# Autodesk Inventor assembly: Frame_Gantry_Carrier_Reverse
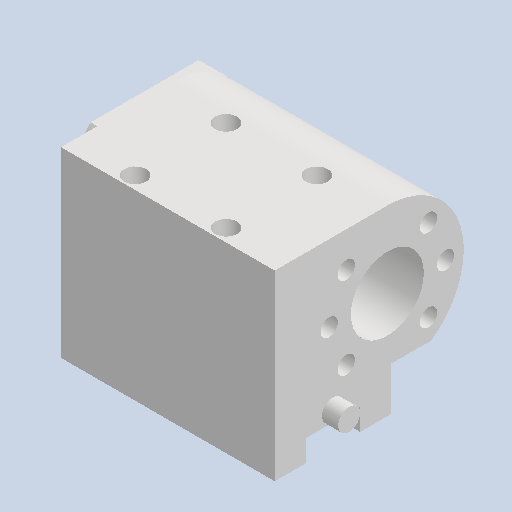
[picture p0: Inventor's stored thumbnail of the model, 512x512]
Saved by Autodesk Inventor 2023 (Build 270158000, 158)
## iProperties
Created: 2022-04-30
Part Number: Frame_Gantry_Carrier_Reverse
Document SubType Name: Assembly
Designer: plebbb
Author: plebbb
## Documents named in this file (4)
- D:\Users\plebbb\Desktop\CNC_Project\Frame_Gantry_Carrier_Reverse.iam
- D:\Users\plebbb\Desktop\CNC_Project\MGN15H-Carrier.ipt
- D:\Users\plebbb\Desktop\CNC_Project\SFU1204-Housing.ipt
- D:\Users\plebbb\Desktop\CNC_Project\X_Axis_Connector.ipt
## Components (3 placed, 3 different names)
1. MGN15H-Carrier:1
2. SFU1204-Housing:1
3. X_Axis_Connector:1
## Relationships (5: Mate 4, Angle 1)
- [Angle] (0 deg): MGN15H-Carrier:1 ↔ SFU1204-Housing:1
- [Mate]: MGN15H-Carrier:1 ↔ SFU1204-Housing:1
- [Mate]: MGN15H-Carrier:1 ↔ X_Axis_Connector:1
- [Mate]: MGN15H-Carrier:1 ↔ X_Axis_Connector:1
- [Mate]: MGN15H-Carrier:1 ↔ X_Axis_Connector:1
